# Autodesk Inventor assembly: connected connectors
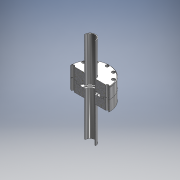
[picture p0: Inventor's stored thumbnail of the model, 180x180]
Saved by Autodesk Inventor 2018 (Build 220112000, 112)
## iProperties
Created: 2019-01-21
Part Number: connected connectors
Document SubType Name: Assembly
Designer: Admin
Author: Admin
## Documents named in this file (3)
- C:\Users\Admin\Documents\Cryostat\CAD\connected connectors.iam
- C:\Users\Admin\Documents\Cryostat\CAD\universal connector male.ipt
- C:\Users\Admin\Documents\Cryostat\CAD\universal connector.ipt
## Components (2 placed, 2 different names)
1. universal connector male:1 — Mate:1, Mate:2
2. universal connector:1 — Mate:1, Mate:2
## Relationships (2: Mate 2)
- Mate:1: universal connector male:1 ↔ universal connector:1
- Mate:2: universal connector male:1 ↔ universal connector:1
